# Autodesk Inventor assembly: Assembly
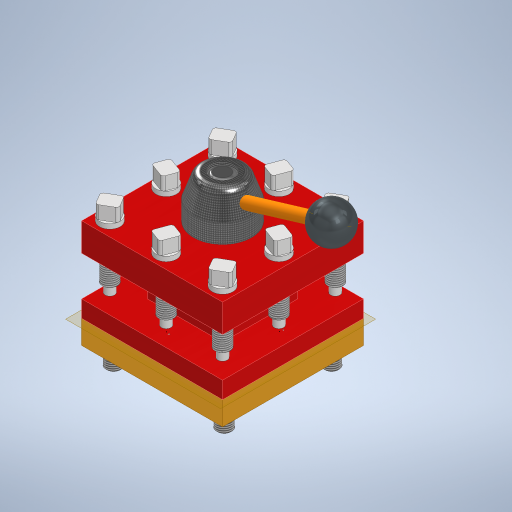
[picture p0: Inventor's stored thumbnail of the model, 512x512]
Saved by Autodesk Inventor 2024 (Build 280153000, 153)
## iProperties
Created: 2023-11-16
Part Number: Assembly
Document SubType Name: Assembly
Designer: Admin
Author: Admin
## Documents named in this file (11)
- C:\Users\Admin\Documents\Inventor\class7.assembly\Assembly.iam
- C:\Users\Admin\Documents\Inventor\class7.assembly\BasePlate.ipt
- C:\Users\Admin\Documents\Inventor\class7.assembly\M16bolt.ipt
- C:\Users\Admin\Documents\Inventor\class7.assembly\spring.ipt
- C:\Users\Admin\Documents\Inventor\class7.assembly\Body.ipt
- C:\Users\Admin\Documents\Inventor\class7.assembly\Stud.ipt
- C:\Users\Admin\Documents\Inventor\class7.assembly\ClampingNut.ipt
- C:\Users\Admin\Documents\Inventor\class7.assembly\Ball.ipt
- C:\Users\Admin\Documents\Inventor\class7.assembly\Handle.ipt
- C:\Users\Admin\Documents\Inventor\class7.assembly\Knob.ipt
- C:\Users\Admin\Documents\Inventor\class7.assembly\SetScrew.ipt
## Components (26 placed, 10 different names)
1. BasePlate:1 — Mate:1, Mate:2, Mate:3, Mate:4, Flush:1, Flush:2, Flush:3, Flush:4, Mate:13, Tangent:2, Mate:16, Flush:15, Flush:16, Insert:2, Flush:17, Flush:18
2. M16bolt:1 — Mate:1, Flush:4
3. M16bolt:2 — Mate:2, Flush:1
4. M16bolt:3 — Mate:3, Flush:2
5. M16bolt:4 — Mate:4, Flush:3
6. Body:1 — Mate:13, Mate:14, Tangent:2, Mate:16, Tangent:3, Mate:17, Mate:21, Mate:22, Mate:23, Mate:24, Flush:17, Flush:18
7. Stud:1 — Mate:14, Tangent:3, Flush:15, Mate:18
8. ClampingNut:1 — Mate:17, Mate:18, Insert:1
9. Handle:1 — Insert:1, Mate:19, Mate:20
10. Knob:1 — Mate:19, Mate:20
11. SetScrew:1 — Mate:21, Mate:22
12. SetScrew:2
13. SetScrew:3
14. SetScrew:4
15. SetScrew:5 — Mate:23, Mate:24
16. SetScrew:6
17. SetScrew:7
18. SetScrew:8
19. Ball:1 — Insert:2
20. Ball:2 — Mate:25
21. Ball:3
22. Ball:4
23. spring:1 — Mate:25
24. spring:2
25. spring:3
26. spring:4
## Component patterns: (4 elements, first: SetScrew:1), (4 elements, first: SetScrew:5), (4 elements, first: Ball:1), (4 elements, first: spring:1)
## Relationships (34: Mate 16, Flush 14, Tangent 2, Insert 2)
- Mate:1: BasePlate:1 ↔ M16bolt:1
- Mate:2: BasePlate:1 ↔ M16bolt:2
- Mate:3: BasePlate:1 ↔ M16bolt:3
- Mate:4: BasePlate:1 ↔ M16bolt:4
- Flush:1: BasePlate:1 ↔ M16bolt:2
- Flush:2: BasePlate:1 ↔ M16bolt:3
- Flush:3: BasePlate:1 ↔ M16bolt:4
- Flush:4: BasePlate:1 ↔ M16bolt:1
- Flush:5 (-7.5 mm)
- Flush:10 (-51.25 mm)
- Flush:11 (69.25 mm)
- Flush:12 (9 mm)
- Flush:13 (52.75 mm)
- Flush:14 (-67.5 mm)
- Mate:13: BasePlate:1 ↔ Body:1
- Mate:14: Body:1 ↔ Stud:1
- Tangent:2: BasePlate:1 ↔ Body:1
- Mate:16 (1 mm): BasePlate:1 ↔ Body:1
- Tangent:3: Body:1 ↔ Stud:1
- Flush:15: BasePlate:1 ↔ Stud:1
- Mate:17: Body:1 ↔ ClampingNut:1
- Mate:18: Stud:1 ↔ ClampingNut:1
- Insert:1: ClampingNut:1 ↔ Handle:1
- Mate:19: Handle:1 ↔ Knob:1
- Mate:20: Handle:1 ↔ Knob:1
- Mate:21: Body:1 ↔ SetScrew:1
- Mate:22: Body:1 ↔ SetScrew:1
- Mate:23: Body:1 ↔ SetScrew:5
- Mate:24: Body:1 ↔ SetScrew:5
- Flush:16 (20 mm): BasePlate:1
- Insert:2: BasePlate:1 ↔ Ball:1
- Mate:25: Ball:2 ↔ spring:1
- Flush:17: BasePlate:1 ↔ Body:1
- Flush:18: BasePlate:1 ↔ Body:1
